# Autodesk Inventor assembly: Assembly6
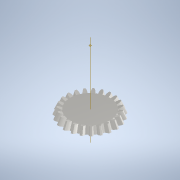
[picture p0: Inventor's stored thumbnail of the model, 180x180]
Saved by Autodesk Inventor 2022 (Build 260153000, 153)
## iProperties
Created: 2022-04-03
Part Number: Assembly6
Document SubType Name: Assembly
Designer: Mlees
Author: Mlees
## Documents named in this file (3)
- C:\Users\Mlees\Desktop\504Engineering\Project_0000\Designs\Design_1\Created_Parts\Assembly6.iam
- C:\Users\Mlees\Desktop\504Engineering\Project_0000\Designs\Design_1\Created_Parts\Plamet_Carrier.ipt
- C:\Users\Mlees\Desktop\504Engineering\Project_0000\Designs\Design_1\Created_Parts\Bevel_Gears\Design Accelerator\Bevel Gear11.ipt
## Components (2 placed, 2 different names)
1. Plamet_Carrier:1 — Rotational:1
2. Bevel Gear1:1 — Rotational:1
## Relationships (1: RevoluteJoint 1)
- Rotational:1 [RevoluteJoint]: Plamet_Carrier:1 ↔ Bevel Gear1:1
